# Autodesk Inventor assembly: Wheel Assembly
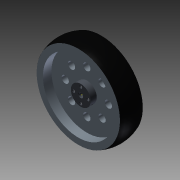
[picture p0: Inventor's stored thumbnail of the model, 180x180]
Saved by Autodesk Inventor 2015 (Build 190159000, 159)
## iProperties
Created: 2015-09-28
Part Number: Wheel Assembly
Document SubType Name: Assembly
Designer: Jing-Chen
Author: Jing-Chen
## Documents named in this file (4)
- C:\Users\Jing-Chen\Desktop\Bionic Hybrids 2016\Bionic-Hybrids\CAD\Drivetrain\Sub-Assemblies\Wheel Assembly.iam
- C:\Users\Jing-Chen\Desktop\Bionic Hybrids 2016\Bionic-Hybrids\Stock\Wheel-Medium(4 in) - 739055.ipt
- C:\Users\Jing-Chen\Desktop\Bionic Hybrids 2016\Bionic-Hybrids\Stock\Shaft Collar-Setscrew, Axle, Mountable - 739172.iam
- C:\Users\Jing-Chen\Desktop\Bionic Hybrids 2016\Bionic-Hybrids\CAD\Drivetrain\Modified Parts\0.75-inch Screw.ipt
## Components (7 placed, 3 different names)
1. Wheel-Medium(4 in) - 739055:1 — Mate:1, Mate:2, Mate:3, Mate:4, Mate:5, Mate:6
2. Shaft Collar-Setscrew, Axle, Mountable - 739172:1 [sub-assembly] — Mate:3, Mate:4, Mate:6, Mate:7, Mate:8, Mate:9, Mate:10, Mate:11, Mate:12, Mate:13, Mate:14
3. Shaft Collar-Setscrew, Axle, Mountable - 739172:2 [sub-assembly] — Mate:1, Mate:2, Mate:5
4. 0.75-inch Screw:1 — Mate:7, Mate:13
5. 0.75-inch Screw:2 — Mate:9, Mate:11
6. 0.75-inch Screw:3 — Mate:8, Mate:12
7. 0.75-inch Screw:4 — Mate:10, Mate:14
## Relationships (14: Mate 14)
- Mate:1: Wheel-Medium(4 in) - 739055:1 ↔ Shaft Collar-Setscrew, Axle, Mountable - 739172:2
- Mate:2: Wheel-Medium(4 in) - 739055:1 ↔ Shaft Collar-Setscrew, Axle, Mountable - 739172:2
- Mate:3: Wheel-Medium(4 in) - 739055:1 ↔ Shaft Collar-Setscrew, Axle, Mountable - 739172:1
- Mate:4: Wheel-Medium(4 in) - 739055:1 ↔ Shaft Collar-Setscrew, Axle, Mountable - 739172:1
- Mate:5: Wheel-Medium(4 in) - 739055:1 ↔ Shaft Collar-Setscrew, Axle, Mountable - 739172:2
- Mate:6: Wheel-Medium(4 in) - 739055:1 ↔ Shaft Collar-Setscrew, Axle, Mountable - 739172:1
- Mate:7: Shaft Collar-Setscrew, Axle, Mountable - 739172:1 ↔ 0.75-inch Screw:1
- Mate:8: Shaft Collar-Setscrew, Axle, Mountable - 739172:1 ↔ 0.75-inch Screw:3
- Mate:9: Shaft Collar-Setscrew, Axle, Mountable - 739172:1 ↔ 0.75-inch Screw:2
- Mate:10: Shaft Collar-Setscrew, Axle, Mountable - 739172:1 ↔ 0.75-inch Screw:4
- Mate:11: Shaft Collar-Setscrew, Axle, Mountable - 739172:1 ↔ 0.75-inch Screw:2
- Mate:12: Shaft Collar-Setscrew, Axle, Mountable - 739172:1 ↔ 0.75-inch Screw:3
- Mate:13: Shaft Collar-Setscrew, Axle, Mountable - 739172:1 ↔ 0.75-inch Screw:1
- Mate:14: Shaft Collar-Setscrew, Axle, Mountable - 739172:1 ↔ 0.75-inch Screw:4
